# Autodesk Inventor assembly: Projekt
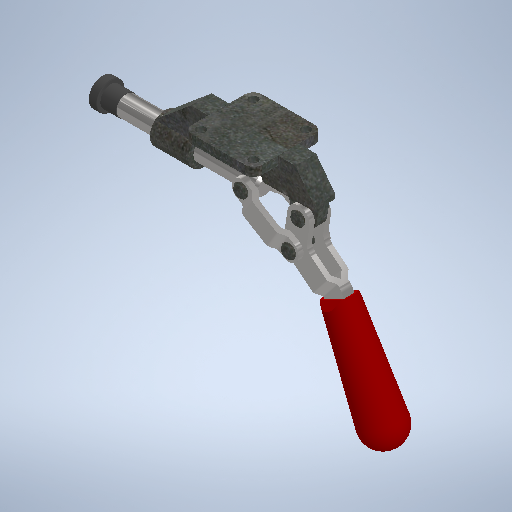
[picture p0: Inventor's stored thumbnail of the model, 512x512]
Saved by Autodesk Inventor 2025.2 (Build 292293000, 293)
## iProperties
Created: 2024-12-01
Part Number: Projekt
Document SubType Name: Assembly
Designer: Marek
Author: Marek
## Documents named in this file (9)
- C:\Users\Marek\Desktop\Chessboard-main\Cad\Projekt.iam
- C:\Users\Marek\Desktop\Chessboard-main\Cad\part1.ipt
- C:\Users\Marek\Desktop\Chessboard-main\Cad\part2.ipt
- C:\Users\Marek\Desktop\Chessboard-main\Cad\part3.ipt
- C:\Users\Marek\Desktop\Chessboard-main\Cad\part4.ipt
- C:\Users\Marek\Desktop\Chessboard-main\Cad\part5.ipt
- C:\Users\Marek\Desktop\Chessboard-main\Cad\part6.ipt
- C:\Users\Marek\Desktop\Chessboard-main\Cad\part7.ipt
- C:\Users\Marek\Documents\Inventor\Content Center Files\R2025\pl-PL\BS EN 22 341  A\ISO 2341 - A - 5 x 10BS EN.ipt
## Components (16 placed, 8 different names)
1. part1:1 — Zestawiające:1, Sztywne:1, Zestawiające:2, Zestawiające:3
2. part2:1 — Zestawiające:2, Zestawiające:3, Zestawiające:5, Zestawiające:6, Zestawiające:8, Zestawiające:9, Sztywne:3, Wstawiające:1, Wstawiające:2, Wstawiające:3, Wstawiające:4
3. part3:1 — Zestawiające:4, Zestawiające:5, Zestawiające:6, Wstawiające:7, Wstawiające:8
4. part4:1 — Sztywne:3
5. part5:1 — Zestawiające:1, Zestawiające:4, Zestawiające:7, Sztywne:2
6. part6:1 — Sztywne:1
7. part7:1 — Sztywne:2
8. part3:2 — Zestawiające:7, Zestawiające:8, Zestawiające:9, Wstawiające:5, Wstawiające:6
9. BS EN 22341 A A - 5 x 10:1 — Wstawiające:1
10. BS EN 22341 A A - 5 x 10:2 — Wstawiające:2
11. BS EN 22341 A A - 5 x 10:3 — Wstawiające:3
12. BS EN 22341 A A - 5 x 10:4 — Wstawiające:4
13. BS EN 22341 A A - 5 x 10:5 — Wstawiające:5
14. BS EN 22341 A A - 5 x 10:6 — Wstawiające:6
15. BS EN 22341 A A - 5 x 10:7 — Wstawiające:7
16. BS EN 22341 A A - 5 x 10:8 — Wstawiające:8
## Relationships (20: Mate 9, Insert 8, WeldJoint 3)
- Zestawiające:1 [Mate]: part1:1 ↔ part5:1
- Sztywne:1 [WeldJoint]: part1:1 ↔ part6:1
- Zestawiające:2 [Mate]: part1:1 ↔ part2:1
- Zestawiające:3 [Mate] (0.175 mm): part1:1 ↔ part2:1
- Zestawiające:4 [Mate]: part3:1 ↔ part5:1
- Zestawiające:5 [Mate]: part2:1 ↔ part3:1
- Zestawiające:6 [Mate]: part2:1 ↔ part3:1
- Zestawiające:7 [Mate]: part5:1 ↔ part3:2
- Zestawiające:8 [Mate]: part2:1 ↔ part3:2
- Zestawiające:9 [Mate]: part2:1 ↔ part3:2
- Sztywne:2 [WeldJoint]: part5:1 ↔ part7:1
- Sztywne:3 [WeldJoint]: part2:1 ↔ part4:1
- Wstawiające:1 [Insert]: part2:1 ↔ BS EN 22341 A A - 5 x 10:1
- Wstawiające:2 [Insert]: part2:1 ↔ BS EN 22341 A A - 5 x 10:2
- Wstawiające:3 [Insert]: part2:1 ↔ BS EN 22341 A A - 5 x 10:3
- Wstawiające:4 [Insert]: part2:1 ↔ BS EN 22341 A A - 5 x 10:4
- Wstawiające:5 [Insert]: part3:2 ↔ BS EN 22341 A A - 5 x 10:5
- Wstawiające:6 [Insert]: part3:2 ↔ BS EN 22341 A A - 5 x 10:6
- Wstawiające:7 [Insert]: part3:1 ↔ BS EN 22341 A A - 5 x 10:7
- Wstawiające:8 [Insert]: part3:1 ↔ BS EN 22341 A A - 5 x 10:8
